# Autodesk Inventor assembly: pelvis_w_motor_fin1_opp
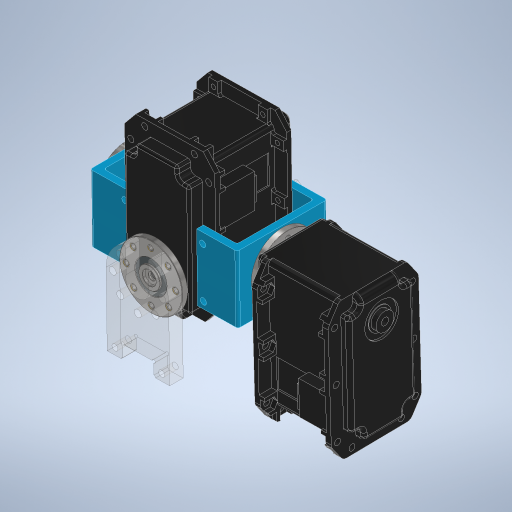
[picture p0: Inventor's stored thumbnail of the model, 512x512]
Saved by Autodesk Inventor 2024 (Build 280153000, 153)
## iProperties
Created: 2024-09-14
Part Number: pelvis_w_motor_fin1_opp
Document SubType Name: Assembly
Designer: jmha0
Author: jmha0
## Documents named in this file (9)
- C:\Users\jmha0\OneDrive\바탕 화면\19th_intern_hjm_fight_robot\Lower_Body\pelvis_w_motor\pelvis_w_motor_fin1_opp.iam
- C:\Users\jmha0\OneDrive\바탕 화면\19th_intern_hjm_fight_robot\Lower_Body\pelvis_w_motor\frame_knee_to_pelvis1.ipt
- C:\Users\jmha0\OneDrive\바탕 화면\19th_intern_hjm_fight_robot\hardware\ROBOTIS(Inventor 2024 ver.)\다이나믹셀\MX-106T+idle.ipt.iam
- C:\Users\jmha0\OneDrive\바탕 화면\19th_intern_hjm_fight_robot\hardware\ROBOTIS(Inventor 2024 ver.)\다이나믹셀\MX-64T.ipt
- C:\Users\jmha0\OneDrive\바탕 화면\19th_intern_hjm_fight_robot\hardware\ROBOTIS(Inventor 2024 ver.)\아이들러\64아이들러.iam
- C:\Users\jmha0\OneDrive\바탕 화면\19th_intern_hjm_fight_robot\hardware\ROBOTIS(Inventor 2024 ver.)\혼\64-106Horn.ipt
- C:\Users\jmha0\OneDrive\바탕 화면\19th_intern_hjm_fight_robot\Lower_Body\pelvis_w_motor\3D_pelvis2.ipt
- C:\Users\jmha0\OneDrive\바탕 화면\19th_intern_hjm_fight_robot\Lower_Body\pelvis_w_motor\3D_pelvis1.ipt
- MX-106T+idle.ipt
## Components (9 placed, 7 different names)
1. frame_knee_to_pelvis1:1
2. MX-106T+idle.ipt:1 [sub-assembly] — 삽입:21, 삽입:22, 삽입:23, 삽입:24, 삽입:25
3. MX-64T:1
4. 64아이들러:1 [sub-assembly]
5. 64-106Horn:1
6. frame_knee_to_pelvis1:2
7. 3D_pelvis2:1 — 삽입:23, 삽입:24
8. 3D_pelvis1:1 — 삽입:21, 삽입:22, 삽입:25
9. 64-106Horn:2
## Relationships (19: Insert 19)
- [Insert] (0.1 mm): MX-106T+idle.ipt:1 ↔ 64-106Horn:1
- [Insert]: frame_knee_to_pelvis1:1 ↔ 64-106Horn:1
- [Insert]: frame_knee_to_pelvis1:1 ↔ 64-106Horn:1
- [Insert]: frame_knee_to_pelvis1:1 ↔ 64-106Horn:1
- [Insert]: frame_knee_to_pelvis1:1 ↔ 64-106Horn:1
- [Insert]: frame_knee_to_pelvis1:1 ↔ 64-106Horn:1
- [Insert]: frame_knee_to_pelvis1:1 ↔ 64-106Horn:1
- [Insert]: MX-106T+idle.ipt:1 ↔ frame_knee_to_pelvis1:2
- [Insert]: MX-106T+idle.ipt:1 ↔ frame_knee_to_pelvis1:2
- [Insert]: MX-106T+idle.ipt:1 ↔ frame_knee_to_pelvis1:2
- [Insert] (0.1 mm): MX-64T:1 ↔ 64-106Horn:2
- [Insert]: 3D_pelvis2:1 ↔ 64-106Horn:2
- [Insert]: 3D_pelvis2:1 ↔ 64-106Horn:2
- [Insert]: 64아이들러:1 ↔ 3D_pelvis1:1
- 삽입:21 [Insert]: MX-106T+idle.ipt:1 ↔ 3D_pelvis1:1
- 삽입:22 [Insert]: MX-106T+idle.ipt:1 ↔ 3D_pelvis1:1
- 삽입:23 [Insert]: MX-106T+idle.ipt:1 ↔ 3D_pelvis2:1
- 삽입:24 [Insert]: MX-106T+idle.ipt:1 ↔ 3D_pelvis2:1
- 삽입:25 [Insert]: MX-106T+idle.ipt:1 ↔ 3D_pelvis1:1
## Named parameters: d16_d17 = 0.1 mm, d17_d18 = 0 mm, d18_d19 = 0 mm
